# Autodesk Inventor assembly: Dispensador
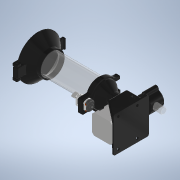
[picture p0: Inventor's stored thumbnail of the model, 180x180]
Saved by Autodesk Inventor 2020.2 (Build 242310000, 310)
## iProperties
Created: 2020-10-21
Part Number: Dispensador
Document SubType Name: Assembly
Designer: JK
Author: JK
## Documents named in this file (15)
- C:\Users\JK\Documents\Inventor\DispensadorPolvo\Dispensador.iam
- C:\Users\JK\Documents\Inventor\DispensadorPolvo\MotorBracket.ipt
- C:\Users\JK\Documents\Inventor\DispensadorPolvo\Tube.ipt
- C:\Users\JK\Documents\Inventor\DispensadorPolvo\StepperMotor.ipt
- C:\Users\JK\Documents\Inventor\DispensadorPolvo\Tornillo.ipt
- C:\Users\JK\Documents\Inventor\DispensadorPolvo\Bearing.ipt
- C:\Users\JK\Documents\Inventor\DispensadorPolvo\BearingHolderInlet.ipt
- C:\Users\JK\Documents\Inventor\DispensadorPolvo\Tube2.ipt
- C:\Users\JK\Documents\Inventor\DispensadorPolvo\Chute.ipt
- C:\Users\JK\Documents\Inventor\DispensadorPolvo\Embudo.ipt
- C:\Users\JK\Documents\Inventor\DispensadorPolvo\Contenedor.ipt
- C:\Users\JK\Documents\Inventor\DispensadorPolvo\Tapacontenedor.ipt
- C:\Users\JK\Documents\Inventor\DispensadorPolvo\vibrator holder.ipt
- C:\Users\JK\Documents\Inventor\DispensadorPolvo\3V DC Electromotor.ipt
- C:\Users\JK\Documents\Inventor\DispensadorPolvo\extra.ipt
## Components (16 placed, 14 different names)
1. MotorBracket:1 — Mate:2, Mate:3, Angle:1, Mate:4, Mate:8, Mate:20, Mate:22, Mate:26
2. Tube:1 — Mate:3, Mate:7, Mate:11, Mate:23
3. StepperMotor:1 — Mate:2, Angle:1, Mate:4, Mate:6, Angle:2
4. Tornillo:1 — Mate:6, Mate:24
5. Bearing:1 — Mate:7, Mate:8, Mate:23
6. Bearing:2 — Mate:11, Mate:17, Mate:19, Mate:24
7. BearingHolderInlet:1 — Mate:17, Mate:19, Mate:21, Mate:22
8. Tube2:1 — Mate:20, Mate:25
9. Tube2:2 — Mate:21
10. Chute:1 — Mate:25, Mate:26, Mate:27, Mate:33
11. Embudo:1 — Mate:27, Mate:28, Mate:30, Angle:2, Mate:31, Mate:32
12. Contenedor:1 — Mate:28, Mate:30
13. Tapacontenedor:1 — Mate:31, Mate:32
14. vibrator holder:1 — Mate:33, Angle:3
15. 3V DC Electromotor:1 — Angle:3, Mate:35
16. extra:1 — Mate:35
## Relationships (26: Mate 23, Angle 3)
- Mate:2: MotorBracket:1 ↔ StepperMotor:1
- Mate:3: MotorBracket:1 ↔ Tube:1
- Angle:1 (0 deg): MotorBracket:1 ↔ StepperMotor:1
- Mate:4: MotorBracket:1 ↔ StepperMotor:1
- Mate:6: StepperMotor:1 ↔ Tornillo:1
- Mate:7: Tube:1 ↔ Bearing:1
- Mate:8: MotorBracket:1 ↔ Bearing:1
- Mate:11: Tube:1 ↔ Bearing:2
- Mate:17: Bearing:2 ↔ BearingHolderInlet:1
- Mate:19: Bearing:2 ↔ BearingHolderInlet:1
- Mate:20: MotorBracket:1 ↔ Tube2:1
- Mate:21: BearingHolderInlet:1 ↔ Tube2:2
- Mate:22: MotorBracket:1 ↔ BearingHolderInlet:1
- Mate:23: Tube:1 ↔ Bearing:1
- Mate:24: Tornillo:1 ↔ Bearing:2
- Mate:25: Tube2:1 ↔ Chute:1
- Mate:26: MotorBracket:1 ↔ Chute:1
- Mate:27: Chute:1 ↔ Embudo:1
- Mate:28: Embudo:1 ↔ Contenedor:1
- Mate:30: Embudo:1 ↔ Contenedor:1
- Angle:2 (0 deg): StepperMotor:1 ↔ Embudo:1
- Mate:31: Embudo:1 ↔ Tapacontenedor:1
- Mate:32 (1 mm): Embudo:1 ↔ Tapacontenedor:1
- Mate:33: Chute:1 ↔ vibrator holder:1
- Angle:3 (0 deg): vibrator holder:1 ↔ 3V DC Electromotor:1
- Mate:35: 3V DC Electromotor:1 ↔ extra:1
